# Autodesk Inventor assembly: Small Continuous Servo
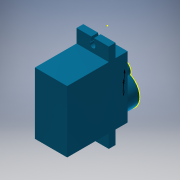
[picture p0: Inventor's stored thumbnail of the model, 180x180]
Saved by Autodesk Inventor 2016 SP2 (Build 200236200, 236)
## iProperties
Created: 2015-07-14
Part Number: Small Continuous Servo
Document SubType Name: Assembly
Designer: Jared
Author: Jared
## Documents named in this file (3)
- E:\Jared\Documents\Inventor\Robotic Hand\Small Continuous Servo.iam
- E:\Jared\Documents\Inventor\Robotic Hand\Small continuous Servo Body.ipt
- E:\Jared\Documents\Inventor\Robotic Hand\Small Continuous Servo Gear.ipt
## Components (2 placed, 2 different names)
1. Small continuous Servo Body:1 — Rotational:1
2. Small Continuous Servo Gear:1 — Rotational:1
## Relationships (1: RevoluteJoint 1)
- Rotational:1 [RevoluteJoint]: Small continuous Servo Body:1 ↔ Small Continuous Servo Gear:1
